# Autodesk Inventor assembly: креплениедатчика
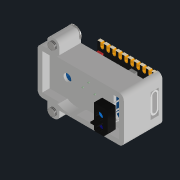
[picture p0: Inventor's stored thumbnail of the model, 180x180]
Saved by Autodesk Inventor 2022 (Build 260153000, 153)
## iProperties
Created: 2025-02-01
Part Number: креплениедатчика
Document SubType Name: Assembly
Designer: it
Author: it
## Documents named in this file (5)
- E:\машина\креплениедатчика.iam
- E:\машина\крепл. датчк.1.ipt
- E:\abuyz lkz vfibyrb\ESP32S3 Super Mini.ipt
- E:\abuyz lkz vfibyrb\TCRT5000.iam
- C:\Users\it\Documents\Inventor\Content Center Files\R2022\ru-RU\GOST 17475-80 (2)\Винт 2.M3-6gx10 ГОСТ 17475-80.ipt
## Components (5 placed, 4 different names)
1. крепл. датчк.1:1 — Совмещение:6, Совмещение:7, Совмещение:8
2. ESP32S3 Super Mini:1
3. Винт 2 ГОСТ 17475-80 M3 x 10:1
4. Винт 2 ГОСТ 17475-80 M3 x 10:2
5. TCRT5000:1 [sub-assembly] — Совмещение:6, Совмещение:7, Совмещение:8
## Relationships (10: Mate 6, Flush 4)
- [Mate]: крепл. датчк.1:1 ↔ ESP32S3 Super Mini:1
- [Flush]: крепл. датчк.1:1 ↔ ESP32S3 Super Mini:1
- [Flush]: крепл. датчк.1:1 ↔ ESP32S3 Super Mini:1
- [Mate]: крепл. датчк.1:1 ↔ Винт 2 ГОСТ 17475-80 M3 x 10:1
- [Mate]: крепл. датчк.1:1 ↔ Винт 2 ГОСТ 17475-80 M3 x 10:2
- [Flush]: крепл. датчк.1:1 ↔ Винт 2 ГОСТ 17475-80 M3 x 10:2
- [Flush]: крепл. датчк.1:1 ↔ Винт 2 ГОСТ 17475-80 M3 x 10:1
- Совмещение:6 [Mate]: крепл. датчк.1:1 ↔ TCRT5000:1
- Совмещение:7 [Mate]: крепл. датчк.1:1 ↔ TCRT5000:1
- Совмещение:8 [Mate] (0.45 mm): крепл. датчк.1:1 ↔ TCRT5000:1
